# Autodesk Inventor assembly: chasis
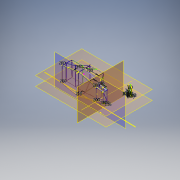
[picture p0: Inventor's stored thumbnail of the model, 180x180]
Saved by Autodesk Inventor 2016 SP1 (Build 200210100, 210)
## iProperties
Created: 2016-06-23
Part Number: chasis
Document SubType Name: Assembly
Designer: asvsf
_SolveAssemblyDoc: Frame Generator Solve Assembly
_Version: 15.0.0
Author: asvsf
## Documents named in this file (7)
- C:\Project\Buggy\chasis.iam
- C:\Project\Buggy\loewr.ipt
- C:\Project\Buggy\chasis\Frame\Frame0001.iam
- C:\Project\Buggy\Suspension\Suspension.iam
- C:\Project\Carv2\suspension_body_001.ipt
- C:\Project\Carv2\suspension_front_hole_upper.ipt
- C:\Project\Buggy\Suspension\upper_arm\Design Accelerator\Bearing1.iam
## Components (9 placed, 6 different names)
1. lower:1
2. Frame0001:1 [sub-assembly] — Mate:1, Mate:2, Flush:1, Flush:2, Mate:7, Mate:8, Flush:3
3. Suspension:2 [sub-assembly]
4. suspension_body_001:1 — Mate:1, Flush:1, Mate:3, Mate:7
5. suspension_body_001:2 — Mate:2, Flush:2, Mate:3
6. suspension_front_hole_upper:1
7. suspension_body_001:3 — Mate:8, Flush:3
8. Bearing:1 [sub-assembly]
9. Bearing:2 [sub-assembly]
## Relationships (8: Mate 5, Flush 3)
- Mate:1: Frame0001:1 ↔ suspension_body_001:1
- Mate:2: Frame0001:1 ↔ suspension_body_001:2
- Flush:1 (-2.5 mm): Frame0001:1 ↔ suspension_body_001:1
- Flush:2 (-2.5 mm): Frame0001:1 ↔ suspension_body_001:2
- Mate:3 (50 mm): suspension_body_001:1 ↔ suspension_body_001:2
- Mate:7 (100 mm): Frame0001:1 ↔ suspension_body_001:1
- Mate:8: Frame0001:1 ↔ suspension_body_001:3
- Flush:3 (-2.5 mm): Frame0001:1 ↔ suspension_body_001:3
